# Autodesk Inventor assembly: ASDSAssembly
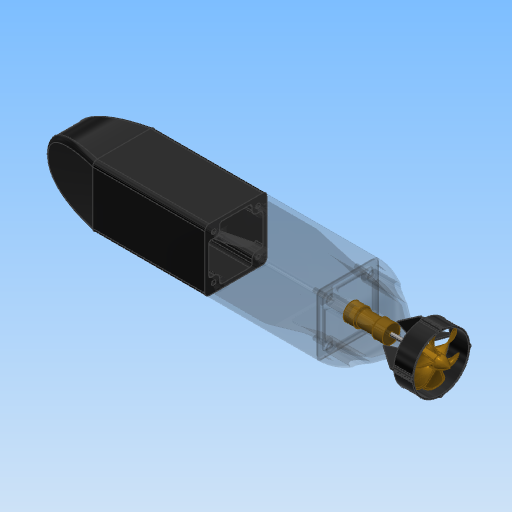
[picture p0: Inventor's stored thumbnail of the model, 512x512]
Saved by Autodesk Inventor 2017 (Build 210142000, 142)
## iProperties
Created: 2017-02-12
Part Number: ASDSAssembly
Document SubType Name: Assembly
Designer: techn
Author: techn
## Documents named in this file (11)
- G:\Projects\Submarine\Submarine-project\CAD\ASDS\ASDSAssembly.iam
- G:\Projects\Submarine\Submarine-project\CAD\ASDS\Fore.ipt
- G:\Projects\Submarine\Submarine-project\CAD\ASDS\MidshipsHullFrontSection.ipt
- G:\Projects\Submarine\Submarine-project\CAD\ASDS\MidshipsHullRearSection.ipt
- G:\Projects\Submarine\Submarine-project\CAD\ASDS\Aft.ipt
- G:\Projects\Submarine\Submarine-project\CAD\common\SleeveBearing2mm.ipt
- G:\Projects\Submarine\Submarine-project\CAD\ASDS\ASDSPropeller.ipt
- G:\Projects\Submarine\Submarine-project\CAD\ASDS\PropShroud.ipt
- G:\Projects\Submarine\Submarine-project\CAD\ASDS\PropShroudSupport.ipt
- G:\Projects\Submarine\Submarine-project\CAD\ASDS\PropShaft.ipt
- G:\Projects\Submarine\Submarine-project\CAD\ASDS\ShaftCoupler.ipt
## Components (13 placed, 10 different names)
1. Fore:1 — Mate:1, Mate:2, Mate:3
2. MidshipsHullFrontSection:1 — Mate:1, Mate:2, Mate:3, Mate:4, Mate:5, Mate:6
3. MidshipsHullRearSection:1 — Mate:4, Mate:5, Mate:6, Mate:7, Mate:8, Mate:9
4. Aft:1 — Mate:7, Mate:8, Mate:9, Mate:10, Flush:1, Mate:12, Mate:14
5. SleeveBearing2mm:1 — Mate:10, Flush:1, Mate:11
6. ASDSPropeller:1 — Mate:11, Mate:12, Mate:13, Mate:23, Mate:24
7. PropShroudSupport:1 — Mate:15, Mate:22, Flush:2
8. PropShroudSupport:2 — Mate:18, Mate:21, Flush:5
9. PropShroudSupport:3 — Mate:16, Mate:19, Flush:3
10. PropShroudSupport:4 — Mate:17, Mate:20, Flush:4
11. PropShroud:1 — Mate:13, Mate:14, Mate:15, Mate:16, Mate:17, Mate:18, Mate:19, Mate:20, Mate:21, Mate:22, Flush:2, Flush:3, Flush:4, Flush:5
12. PropShaft:1 — Mate:23, Mate:24, Mate:25, Mate:26
13. ShaftCoupler:1 — Mate:25, Mate:26
## Relationships (31: Mate 26, Flush 5)
- Mate:1: Fore:1 ↔ MidshipsHullFrontSection:1
- Mate:2: Fore:1 ↔ MidshipsHullFrontSection:1
- Mate:3: Fore:1 ↔ MidshipsHullFrontSection:1
- Mate:4: MidshipsHullFrontSection:1 ↔ MidshipsHullRearSection:1
- Mate:5: MidshipsHullFrontSection:1 ↔ MidshipsHullRearSection:1
- Mate:6: MidshipsHullFrontSection:1 ↔ MidshipsHullRearSection:1
- Mate:7: MidshipsHullRearSection:1 ↔ Aft:1
- Mate:8: MidshipsHullRearSection:1 ↔ Aft:1
- Mate:9: MidshipsHullRearSection:1 ↔ Aft:1
- Mate:10: Aft:1 ↔ SleeveBearing2mm:1
- Flush:1: Aft:1 ↔ SleeveBearing2mm:1
- Mate:11: SleeveBearing2mm:1 ↔ ASDSPropeller:1
- Mate:12 (0.7937 mm): Aft:1 ↔ ASDSPropeller:1
- Mate:13: ASDSPropeller:1 ↔ PropShroud:1
- Mate:14: Aft:1 ↔ PropShroud:1
- Mate:15 (0.0635 mm): PropShroudSupport:1 ↔ PropShroud:1
- Mate:16 (0.0635 mm): PropShroudSupport:3 ↔ PropShroud:1
- Mate:17 (0.0635 mm): PropShroudSupport:4 ↔ PropShroud:1
- Mate:18 (0.0635 mm): PropShroudSupport:2 ↔ PropShroud:1
- Mate:19: PropShroudSupport:3 ↔ PropShroud:1
- Mate:20: PropShroudSupport:4 ↔ PropShroud:1
- Mate:21: PropShroudSupport:2 ↔ PropShroud:1
- Mate:22: PropShroudSupport:1 ↔ PropShroud:1
- Flush:2: PropShroudSupport:1 ↔ PropShroud:1
- Flush:3: PropShroudSupport:3 ↔ PropShroud:1
- Flush:4: PropShroudSupport:4 ↔ PropShroud:1
- Flush:5: PropShroudSupport:2 ↔ PropShroud:1
- Mate:23: ASDSPropeller:1 ↔ PropShaft:1
- Mate:24: ASDSPropeller:1 ↔ PropShaft:1
- Mate:25: PropShaft:1 ↔ ShaftCoupler:1
- Mate:26 (-6.35 mm): PropShaft:1 ↔ ShaftCoupler:1
